# Autodesk Inventor assembly: 810004_X1X
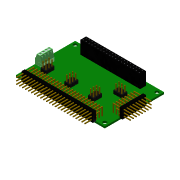
[picture p0: Inventor's stored thumbnail of the model, 180x180]
Saved by Autodesk Inventor 2015 (Build 190159000, 159)
## iProperties
Created: 2014-08-28
Part Number: 810004_X1X
Document SubType Name: Assembly
Designer: david
Author: david
## Documents named in this file (6)
- C:\SharedDrive\Dropbox\FAST Robotics\Products\818004_Power Shield\MECH\810004_Power Shield\810004_X1X.iam
- C:\SharedDrive\Dropbox\FAST Robotics\Products\818004_Power Shield\MECH\810004_Power Shield\810004_XXX.iam
- C:\SharedDrive\Dropbox\FAST Robotics\Products\818004_Power Shield\MECH\810004_Power Shield\SERVO4_RAx8.iam
- C:\SharedDrive\Dropbox\FAST Robotics\Products\818004_Power Shield\MECH\810004_Power Shield\SERVO1_RAx8.iam
- C:\SharedDrive\Dropbox\FAST Robotics\Products\818004_Power Shield\MECH\810004_Power Shield\SERVO2_RAx8.iam
- C:\SharedDrive\Dropbox\FAST Robotics\Products\818004_Power Shield\MECH\810004_Power Shield\SERVO3_RAx8.iam
## Components (5 placed, 5 different names)
1. 810004_XXX:1 [sub-assembly] — Mate:1, Mate:2, Mate:3, Mate:4, Mate:5, Flush:1, Mate:6, Flush:2, Mate:7, Flush:3, Mate:8, Flush:4, Flush:5, Flush:6, Flush:7
2. SERVO4_RAx8:1 [sub-assembly] — Mate:1, Mate:8, Flush:4
3. SERVO1_RAx8:1 [sub-assembly] — Mate:3, Mate:5, Flush:1
4. SERVO2_RAx8:1 [sub-assembly] — Mate:4, Mate:6, Flush:2
5. SERVO3_RAx8:1 [sub-assembly] — Mate:2, Mate:7, Flush:3
## Relationships (15: Mate 8, Flush 7)
- Mate:1: 810004_XXX:1 ↔ SERVO4_RAx8:1
- Mate:2: 810004_XXX:1 ↔ SERVO3_RAx8:1
- Mate:3: 810004_XXX:1 ↔ SERVO1_RAx8:1
- Mate:4: 810004_XXX:1 ↔ SERVO2_RAx8:1
- Mate:5: 810004_XXX:1 ↔ SERVO1_RAx8:1
- Flush:1 (7.62 mm): 810004_XXX:1 ↔ SERVO1_RAx8:1
- Mate:6: 810004_XXX:1 ↔ SERVO2_RAx8:1
- Flush:2 (28.194 mm): 810004_XXX:1 ↔ SERVO2_RAx8:1
- Mate:7: 810004_XXX:1 ↔ SERVO3_RAx8:1
- Flush:3 (7.62 mm): 810004_XXX:1 ↔ SERVO3_RAx8:1
- Mate:8: 810004_XXX:1 ↔ SERVO4_RAx8:1
- Flush:4 (12.7 mm): 810004_XXX:1 ↔ SERVO4_RAx8:1
- Flush:5: 810004_XXX:1
- Flush:6: 810004_XXX:1
- Flush:7: 810004_XXX:1
